# Autodesk Inventor assembly: Base
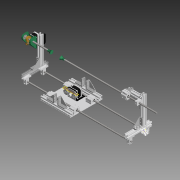
[picture p0: Inventor's stored thumbnail of the model, 180x180]
Saved by Autodesk Inventor 2015 (Build 190159000, 159)
## iProperties
Created: 2015-02-24
Part Number: Base
Document SubType Name: Assembly
Designer: Andrew
Author: Andrew
## Documents named in this file (30)
- C:\Users\pltwe4\Documents\model\Base.iam
- C:\Users\pltwe4\Documents\model\Linear Bearing Platform Small.ipt
- C:\Users\pltwe4\Documents\model\Base Plate.ipt
- C:\Users\pltwe4\Documents\model\NEMA 17 Stepper.ipt
- C:\Users\pltwe4\Documents\model\GT2 Pulley.ipt
- C:\Users\pltwe4\Documents\model\Stepper Motor Mount.ipt
- C:\Users\pltwe4\Documents\model\MainRod.ipt
- C:\Users\pltwe4\Documents\model\Linear Rail Shaft Guide.ipt
- C:\Users\pltwe4\Documents\model\Spur Gear.ipt
- C:\Users\pltwe4\Documents\model\Worm Gear.ipt
- C:\Users\pltwe4\Documents\model\20x20 Slotted Extrusion Arm.ipt
- C:\Users\pltwe4\Documents\model\20x20 Slotted Extrusion Tower.ipt
- C:\Users\pltwe4\Documents\model\Corner Brace.ipt
- C:\Users\pltwe4\Documents\model\Worm Gear Box.ipt
- C:\Users\pltwe4\Documents\model\Bearing.ipt
- C:\Users\pltwe4\Documents\model\20x20 Slotted Extrusion Stationary Arm.ipt
- C:\Users\pltwe4\Documents\model\Clamp Rod.ipt
- C:\Users\pltwe4\Documents\model\Rotational Rod.ipt
- C:\Users\pltwe4\Documents\model\20x20 Slotted Extrusion Base.ipt
- C:\Users\pltwe4\Documents\model\20x20 Slotted Extrusion Source Bracket.ipt
- C:\Users\pltwe4\Documents\model\Cover.ipt
- C:\Users\pltwe4\Documents\model\X-Ray Tube Assy.ipt.iam
- C:\Users\pltwe4\Documents\model\Hand.ipt
- C:\Users\pltwe4\Documents\model\Linear Bearing Adapter Arm.ipt
- C:\Users\pltwe4\Documents\model\20x20 Slotted Extrusion Base2Plate.ipt
- C:\Users\pltwe4\Documents\model\Corner Brace_MIR.ipt
- C:\Users\pltwe4\Documents\model\Stepper Atachments.ipt
- C:\Users\pltwe4\Documents\model\Stepper Cap.ipt
- C:\Users\pltwe4\Documents\model\Belt Clamp.ipt
- X-Ray Tube Assy.ipt
## Components (57 placed, 28 different names)
1. Linear Bearing Platform Small:1 — Flush:5, Mate:7, Flush:9, Flush:11
2. Linear Bearing Platform Small:2 — Flush:4, Flush:5, Flush:6, Mate:6, Angle:2, Flush:8, Flush:10
3. Linear Bearing Platform Small:3 — Flush:4, Mate:8, Flush:8
4. Linear Bearing Platform Small:4 — Flush:6, Mate:1, Mate:9, Angle:3, Flush:9
5. Base Plate:1 — Flush:1, Flush:2, Flush:3, Mate:1, Angle:2, Angle:3, Flush:10, Flush:11, Flush:40, Flush:42, Mate:123, Flush:43, Mate:153, Flush:56, Flush:57, Flush:58, Mate:172
6. GT2 Pulley:1 — Mate:22, Mate:166, Mate:170
7. MainRod:1 — Mate:6, Mate:7, Mate:10, Flush:16, Mate:12, Flush:24
8. MainRod:2 — Mate:8, Mate:9, Mate:11, Flush:16, Mate:13, Flush:23
9. Linear Rail Shaft Guide:1 — Mate:10, Flush:14, Flush:15, Flush:24, Flush:53
10. Linear Rail Shaft Guide:2 — Mate:11, Flush:14, Flush:15, Flush:31, Mate:47, Mate:48, Flush:52
11. Linear Rail Shaft Guide:3 — Mate:12
12. Linear Rail Shaft Guide:4 — Mate:13, Flush:23, Flush:32, Mate:49, Mate:50
13. Spur Gear:1 — Tangent:1, Mate:44, Mate:46, Angle:5, Mate:87, Mate:99
14. Stepper Motor Mount:2 — Mate:40, Mate:41, Mate:42, Angle:5, Mate:53, Mate:54, Mate:55, Mate:79
15. Worm Gear:1 — Mate:27, Mate:28, Tangent:1, Mate:44, Mate:46, Mate:80
16. NEMA 17 Stepper:2 — Mate:27, Mate:28, Mate:40, Mate:41, Mate:42, Mate:81
17. 20x20 Slotted Extrusion Arm:1 — Flush:31, Mate:47, Mate:48, Mate:52, Flush:34, Mate:66, Mate:68, Mate:70, Mate:72, Mate:100, Flush:52, Flush:53
18. 20x20 Slotted Extrusion Tower:1 — Mate:52, Flush:34, Mate:53, Mate:54, Mate:55, Mate:65, Mate:67, Mate:69, Mate:71
19. 20x20 Slotted Extrusion Arm:2 — Flush:32, Mate:49, Mate:50, Mate:51, Flush:33, Mate:57, Mate:58, Mate:63, Mate:64, Flush:62, Mate:187
20. 20x20 Slotted Extrusion Tower:2 — Mate:51, Flush:33, Mate:59, Mate:60, Mate:61, Mate:62, Angle:7, Mate:88, Mate:89, Mate:90, Flush:35, Flush:36, Mate:92, Mate:95
21. Corner Brace:1 — Mate:69, Mate:70, Mate:71, Mate:72
22. Corner Brace:2 — Mate:65, Mate:66, Mate:67, Mate:68
23. Corner Brace:3 — Mate:57, Mate:58, Mate:59, Mate:60
24. Corner Brace:4 — Mate:61, Mate:62, Mate:63, Mate:64
25. Linear Bearing Platform Small:5 — Mate:86, Angle:6, Mate:87, Mate:91, Mate:93, Flush:51, Mate:149, Mate:150
26. Linear Rail Shaft Guide:5 — Mate:86, Angle:6, Angle:7, Mate:88, Mate:89, Mate:90, Flush:35, Mate:91, Flush:50
27. Worm Gear Box:1 — Mate:79, Mate:80, Mate:81, Mate:82, Mate:84, Flush:37
28. Bearing:1 — Mate:82
29. Bearing:2 — Mate:84
30. 20x20 Slotted Extrusion Stationary Arm:1 — Flush:36, Mate:92, Mate:93, Mate:94, Mate:96, Mate:97
31. Corner Brace:5 — Mate:94, Mate:95, Mate:96, Mate:97
32. Clamp Rod:1 — Mate:98, Flush:50, Mate:147, Mate:152
33. Rotational Rod:1 — Mate:98, Mate:99, Flush:37, Mate:100, Mate:146, Mate:148
34. 20x20 Slotted Extrusion Base:1 — Symmetry:2, Flush:39, Flush:40, Mate:135, Mate:137, Flush:59, Mate:155, Mate:157, Mate:158, Mate:162
35. 20x20 Slotted Extrusion Base:2 — Symmetry:2, Flush:39, Mate:107, Flush:41, Mate:134, Flush:59, Mate:154, Mate:160, Mate:161, Mate:163
36. 20x20 Slotted Extrusion Source Bracket:1 — Mate:107, Flush:41, Mate:140, Mate:141, Mate:142, Mate:143, Mate:144, Mate:155
37. Cover:1 — Flush:42, Mate:123, Flush:43
38. Corner Brace:6 — Mate:135, Flush:48, Flush:49, Mate:137
39. Corner Brace:7 — Mate:134, Flush:48, Flush:49, Mate:144
40. X-Ray Tube Assy.ipt:1 [sub-assembly] — Mate:140, Mate:141, Mate:142, Mate:143
41. Hand:1 — Mate:145, Mate:146, Mate:148
42. Hand:2 — Mate:145, Mate:147
43. Linear Bearing Adapter Arm:1 — Flush:51, Mate:149, Mate:150
44. 20x20 Slotted Extrusion Base2Plate:1 — Flush:54, Mate:153, Flush:55, Flush:58, Mate:154, Mate:159, Mate:164, Flush:63
45. 20x20 Slotted Extrusion Base2Plate:2 — Flush:54, Flush:55, Flush:56, Flush:57, Mate:156, Mate:165, Angle:8
46. Corner Brace:8 — Mate:156, Mate:157, Mate:158, Flush:61
47. Corner Brace:9 — Mate:159, Mate:160, Mate:161, Flush:60
48. Corner Brace_MIR:1 — Flush:61, Mate:162, Mate:165
49. Corner Brace_MIR:2 — Flush:60, Mate:163, Mate:164
50. NEMA 17 Stepper:3 — Mate:166, Mate:169, Mate:173, Mate:174, Mate:175, Mate:186, Flush:63
51. Stepper Atachments:1 — Mate:169, Mate:170, Mate:176, Mate:177, Angle:8, Mate:178, Mate:180, Mate:181, Mate:183, Mate:184, Mate:185, Angle:9
52. Stepper Motor Mount:3 — Mate:172, Mate:173, Mate:174, Mate:175, Mate:176, Mate:177
53. Stepper Cap:1 — Mate:178, Mate:179, Mate:181
54. Bearing:3 — Mate:179, Mate:180
55. Stepper Cap:2 — Mate:185
56. Bearing:4 — Mate:183, Mate:184, Tangent:2
57. Belt Clamp:1 — Flush:62, Mate:187
## Relationships (166: Mate 111, Flush 45, Angle 7, Tangent 2, Symmetry 1)
- Flush:1: Base Plate:1
- Flush:2: Base Plate:1
- Flush:3: Base Plate:1
- Flush:4: Linear Bearing Platform Small:2 ↔ Linear Bearing Platform Small:3
- Flush:5: Linear Bearing Platform Small:1 ↔ Linear Bearing Platform Small:2
- Flush:6: Linear Bearing Platform Small:2 ↔ Linear Bearing Platform Small:4
- Mate:1: Linear Bearing Platform Small:4 ↔ Base Plate:1
- Mate:6: Linear Bearing Platform Small:2 ↔ MainRod:1
- Mate:7: Linear Bearing Platform Small:1 ↔ MainRod:1
- Mate:8: Linear Bearing Platform Small:3 ↔ MainRod:2
- Mate:9: Linear Bearing Platform Small:4 ↔ MainRod:2
- Mate:10: MainRod:1 ↔ Linear Rail Shaft Guide:1
- Mate:11: MainRod:2 ↔ Linear Rail Shaft Guide:2
- Angle:2 (0 deg): Linear Bearing Platform Small:2 ↔ Base Plate:1
- Angle:3 (0 deg): Linear Bearing Platform Small:4 ↔ Base Plate:1
- Flush:8: Linear Bearing Platform Small:2 ↔ Linear Bearing Platform Small:3
- Flush:9: Linear Bearing Platform Small:1 ↔ Linear Bearing Platform Small:4
- Flush:10 (5 mm): Linear Bearing Platform Small:2 ↔ Base Plate:1
- Flush:11 (5 mm): Linear Bearing Platform Small:1 ↔ Base Plate:1
- Flush:14: Linear Rail Shaft Guide:1 ↔ Linear Rail Shaft Guide:2
- Flush:15: Linear Rail Shaft Guide:1 ↔ Linear Rail Shaft Guide:2
- Flush:16: MainRod:1 ↔ MainRod:2
- [Flush]: Linear Rail Shaft Guide:3 ↔ Linear Rail Shaft Guide:4
- [Flush]: Linear Rail Shaft Guide:3 ↔ Linear Rail Shaft Guide:4
- Mate:12: MainRod:1 ↔ Linear Rail Shaft Guide:3
- Mate:13: MainRod:2 ↔ Linear Rail Shaft Guide:4
- Flush:23 (5 mm): MainRod:2 ↔ Linear Rail Shaft Guide:4
- Flush:24 (5 mm): MainRod:1 ↔ Linear Rail Shaft Guide:1
- Mate:22: GT2 Pulley:1
- Mate:27: Worm Gear:1 ↔ NEMA 17 Stepper:2
- Mate:28 (3 mm): Worm Gear:1 ↔ NEMA 17 Stepper:2
- Mate:40: Stepper Motor Mount:2 ↔ NEMA 17 Stepper:2
- Mate:41: Stepper Motor Mount:2 ↔ NEMA 17 Stepper:2
- Mate:42: Stepper Motor Mount:2 ↔ NEMA 17 Stepper:2
- Tangent:1: Spur Gear:1 ↔ Worm Gear:1
- Mate:44: Spur Gear:1 ↔ Worm Gear:1
- Mate:46: Spur Gear:1 ↔ Worm Gear:1
- Angle:5 (0 deg): Spur Gear:1 ↔ Stepper Motor Mount:2
- Flush:31: Linear Rail Shaft Guide:2 ↔ 20x20 Slotted Extrusion Arm:1
- Mate:47: Linear Rail Shaft Guide:2 ↔ 20x20 Slotted Extrusion Arm:1
- Mate:48: Linear Rail Shaft Guide:2 ↔ 20x20 Slotted Extrusion Arm:1
- Flush:32: Linear Rail Shaft Guide:4 ↔ 20x20 Slotted Extrusion Arm:2
- Mate:49: Linear Rail Shaft Guide:4 ↔ 20x20 Slotted Extrusion Arm:2
- Mate:50: Linear Rail Shaft Guide:4 ↔ 20x20 Slotted Extrusion Arm:2
- Mate:51: 20x20 Slotted Extrusion Arm:2 ↔ 20x20 Slotted Extrusion Tower:2
- Flush:33: 20x20 Slotted Extrusion Arm:2 ↔ 20x20 Slotted Extrusion Tower:2
- Mate:52: 20x20 Slotted Extrusion Arm:1 ↔ 20x20 Slotted Extrusion Tower:1
- Flush:34: 20x20 Slotted Extrusion Arm:1 ↔ 20x20 Slotted Extrusion Tower:1
- Mate:53: Stepper Motor Mount:2 ↔ 20x20 Slotted Extrusion Tower:1
- Mate:54: Stepper Motor Mount:2 ↔ 20x20 Slotted Extrusion Tower:1
- Mate:55: Stepper Motor Mount:2 ↔ 20x20 Slotted Extrusion Tower:1
- Mate:57: 20x20 Slotted Extrusion Arm:2 ↔ Corner Brace:3
- Mate:58: 20x20 Slotted Extrusion Arm:2 ↔ Corner Brace:3
- Mate:59: 20x20 Slotted Extrusion Tower:2 ↔ Corner Brace:3
- Mate:60: 20x20 Slotted Extrusion Tower:2 ↔ Corner Brace:3
- Mate:61: 20x20 Slotted Extrusion Tower:2 ↔ Corner Brace:4
- Mate:62: 20x20 Slotted Extrusion Tower:2 ↔ Corner Brace:4
- Mate:63: 20x20 Slotted Extrusion Arm:2 ↔ Corner Brace:4
- Mate:64: 20x20 Slotted Extrusion Arm:2 ↔ Corner Brace:4
- Mate:65: 20x20 Slotted Extrusion Tower:1 ↔ Corner Brace:2
- Mate:66: 20x20 Slotted Extrusion Arm:1 ↔ Corner Brace:2
- Mate:67: 20x20 Slotted Extrusion Tower:1 ↔ Corner Brace:2
- Mate:68: 20x20 Slotted Extrusion Arm:1 ↔ Corner Brace:2
- Mate:69: 20x20 Slotted Extrusion Tower:1 ↔ Corner Brace:1
- Mate:70: 20x20 Slotted Extrusion Arm:1 ↔ Corner Brace:1
- Mate:71: 20x20 Slotted Extrusion Tower:1 ↔ Corner Brace:1
- Mate:72: 20x20 Slotted Extrusion Arm:1 ↔ Corner Brace:1
- Mate:79: Stepper Motor Mount:2 ↔ Worm Gear Box:1
- Mate:80: Worm Gear:1 ↔ Worm Gear Box:1
- Mate:81: NEMA 17 Stepper:2 ↔ Worm Gear Box:1
- Mate:82: Worm Gear Box:1 ↔ Bearing:1
- Mate:84: Worm Gear Box:1 ↔ Bearing:2
- Mate:86: Linear Bearing Platform Small:5 ↔ Linear Rail Shaft Guide:5
- Angle:6 (0 deg): Linear Bearing Platform Small:5 ↔ Linear Rail Shaft Guide:5
- Angle:7 (0 deg): 20x20 Slotted Extrusion Tower:2 ↔ Linear Rail Shaft Guide:5
- Mate:87: Spur Gear:1 ↔ Linear Bearing Platform Small:5
- Mate:88: 20x20 Slotted Extrusion Tower:2 ↔ Linear Rail Shaft Guide:5
- Mate:89: 20x20 Slotted Extrusion Tower:2 ↔ Linear Rail Shaft Guide:5
- Mate:90: 20x20 Slotted Extrusion Tower:2 ↔ Linear Rail Shaft Guide:5
- Flush:35 (-5 mm): 20x20 Slotted Extrusion Tower:2 ↔ Linear Rail Shaft Guide:5
- Mate:91 (50 mm): Linear Bearing Platform Small:5 ↔ Linear Rail Shaft Guide:5
- Flush:36: 20x20 Slotted Extrusion Tower:2 ↔ 20x20 Slotted Extrusion Stationary Arm:1
- Mate:92: 20x20 Slotted Extrusion Tower:2 ↔ 20x20 Slotted Extrusion Stationary Arm:1
- Mate:93: Linear Bearing Platform Small:5 ↔ 20x20 Slotted Extrusion Stationary Arm:1
- Mate:94: 20x20 Slotted Extrusion Stationary Arm:1 ↔ Corner Brace:5
- Mate:95: 20x20 Slotted Extrusion Tower:2 ↔ Corner Brace:5
- Mate:96: 20x20 Slotted Extrusion Stationary Arm:1 ↔ Corner Brace:5
- Mate:97: 20x20 Slotted Extrusion Stationary Arm:1 ↔ Corner Brace:5
- Mate:98: Clamp Rod:1 ↔ Rotational Rod:1
- Mate:99: Spur Gear:1 ↔ Rotational Rod:1
- Flush:37 (-5 mm): Worm Gear Box:1 ↔ Rotational Rod:1
- Mate:100: 20x20 Slotted Extrusion Arm:1 ↔ Rotational Rod:1
- Symmetry:2: 20x20 Slotted Extrusion Base:1 ↔ 20x20 Slotted Extrusion Base:2
- Flush:39: 20x20 Slotted Extrusion Base:1 ↔ 20x20 Slotted Extrusion Base:2
- Flush:40: Base Plate:1 ↔ 20x20 Slotted Extrusion Base:1
- Mate:107: 20x20 Slotted Extrusion Base:2 ↔ 20x20 Slotted Extrusion Source Bracket:1
- Flush:41: 20x20 Slotted Extrusion Base:2 ↔ 20x20 Slotted Extrusion Source Bracket:1
- Flush:42: Base Plate:1 ↔ Cover:1
- Mate:123: Base Plate:1 ↔ Cover:1
- Flush:43: Base Plate:1 ↔ Cover:1
- Mate:134: 20x20 Slotted Extrusion Base:2 ↔ Corner Brace:7
- Mate:135: 20x20 Slotted Extrusion Base:1 ↔ Corner Brace:6
- Flush:48: Corner Brace:6 ↔ Corner Brace:7
- Flush:49: Corner Brace:6 ↔ Corner Brace:7
- Mate:137: 20x20 Slotted Extrusion Base:1 ↔ Corner Brace:6
- Mate:140: 20x20 Slotted Extrusion Source Bracket:1 ↔ X-Ray Tube Assy.ipt:1
- Mate:141: 20x20 Slotted Extrusion Source Bracket:1 ↔ X-Ray Tube Assy.ipt:1
- Mate:142: 20x20 Slotted Extrusion Source Bracket:1 ↔ X-Ray Tube Assy.ipt:1
- Mate:143: 20x20 Slotted Extrusion Source Bracket:1 ↔ X-Ray Tube Assy.ipt:1
- Mate:144: 20x20 Slotted Extrusion Source Bracket:1 ↔ Corner Brace:7
- Flush:50 (100 mm): Linear Rail Shaft Guide:5 ↔ Clamp Rod:1
- Mate:145: Hand:1 ↔ Hand:2
- Mate:146: Rotational Rod:1 ↔ Hand:1
- Mate:147: Clamp Rod:1 ↔ Hand:2
- Mate:148: Rotational Rod:1 ↔ Hand:1
- Flush:51: Linear Bearing Platform Small:5 ↔ Linear Bearing Adapter Arm:1
- Mate:149: Linear Bearing Platform Small:5 ↔ Linear Bearing Adapter Arm:1
- Mate:150: Linear Bearing Platform Small:5 ↔ Linear Bearing Adapter Arm:1
- Flush:52: Linear Rail Shaft Guide:2 ↔ 20x20 Slotted Extrusion Arm:1
- Flush:53: Linear Rail Shaft Guide:1 ↔ 20x20 Slotted Extrusion Arm:1
- Mate:152: Clamp Rod:1
- Flush:54: 20x20 Slotted Extrusion Base2Plate:1 ↔ 20x20 Slotted Extrusion Base2Plate:2
- Mate:153: Base Plate:1 ↔ 20x20 Slotted Extrusion Base2Plate:1
- Flush:55: 20x20 Slotted Extrusion Base2Plate:1 ↔ 20x20 Slotted Extrusion Base2Plate:2
- Flush:56: Base Plate:1 ↔ 20x20 Slotted Extrusion Base2Plate:2
- Flush:57: Base Plate:1 ↔ 20x20 Slotted Extrusion Base2Plate:2
- Flush:58: Base Plate:1 ↔ 20x20 Slotted Extrusion Base2Plate:1
- Flush:59: 20x20 Slotted Extrusion Base:1 ↔ 20x20 Slotted Extrusion Base:2
- Mate:154: 20x20 Slotted Extrusion Base:2 ↔ 20x20 Slotted Extrusion Base2Plate:1
- Mate:155: 20x20 Slotted Extrusion Base:1 ↔ 20x20 Slotted Extrusion Source Bracket:1
- Mate:156: 20x20 Slotted Extrusion Base2Plate:2 ↔ Corner Brace:8
- Mate:157: 20x20 Slotted Extrusion Base:1 ↔ Corner Brace:8
- Mate:158: 20x20 Slotted Extrusion Base:1 ↔ Corner Brace:8
- Mate:159: 20x20 Slotted Extrusion Base2Plate:1 ↔ Corner Brace:9
- Mate:160: 20x20 Slotted Extrusion Base:2 ↔ Corner Brace:9
- Mate:161: 20x20 Slotted Extrusion Base:2 ↔ Corner Brace:9
- Flush:60: Corner Brace:9 ↔ Corner Brace_MIR:2
- Flush:61: Corner Brace:8 ↔ Corner Brace_MIR:1
- Mate:162: 20x20 Slotted Extrusion Base:1 ↔ Corner Brace_MIR:1
- Mate:163: 20x20 Slotted Extrusion Base:2 ↔ Corner Brace_MIR:2
- Mate:164: 20x20 Slotted Extrusion Base2Plate:1 ↔ Corner Brace_MIR:2
- Mate:165: 20x20 Slotted Extrusion Base2Plate:2 ↔ Corner Brace_MIR:1
- Mate:166: GT2 Pulley:1 ↔ NEMA 17 Stepper:3
- Mate:169: NEMA 17 Stepper:3 ↔ Stepper Atachments:1
- Mate:170: GT2 Pulley:1 ↔ Stepper Atachments:1
- Mate:172: Base Plate:1 ↔ Stepper Motor Mount:3
- Mate:173: NEMA 17 Stepper:3 ↔ Stepper Motor Mount:3
- Mate:174: NEMA 17 Stepper:3 ↔ Stepper Motor Mount:3
- Mate:175: NEMA 17 Stepper:3 ↔ Stepper Motor Mount:3
- Mate:176: Stepper Atachments:1 ↔ Stepper Motor Mount:3
- Mate:177: Stepper Atachments:1 ↔ Stepper Motor Mount:3
- Angle:8 (0 deg): 20x20 Slotted Extrusion Base2Plate:2 ↔ Stepper Atachments:1
- Mate:178: Stepper Atachments:1 ↔ Stepper Cap:1
- Mate:179: Stepper Cap:1 ↔ Bearing:3
- Mate:180: Stepper Atachments:1 ↔ Bearing:3
- Mate:181: Stepper Atachments:1 ↔ Stepper Cap:1
- [Mate]: Stepper Cap:2 ↔ Bearing:4
- Mate:183: Stepper Atachments:1 ↔ Bearing:4
- Mate:184: Stepper Atachments:1 ↔ Bearing:4
- Mate:185: Stepper Atachments:1 ↔ Stepper Cap:2
- Flush:62: 20x20 Slotted Extrusion Arm:2 ↔ Belt Clamp:1
- Mate:186: NEMA 17 Stepper:3
- Flush:63 (50 mm): 20x20 Slotted Extrusion Base2Plate:1 ↔ NEMA 17 Stepper:3
- Mate:187: 20x20 Slotted Extrusion Arm:2 ↔ Belt Clamp:1
- Angle:9 (0 deg): Stepper Atachments:1
- Tangent:2: Bearing:4
## Named parameters: d31_d27 = 0 mm, d32_d28 = 0 mm, d285_d282 = 0 mm
